# Autodesk Inventor assembly: PBM
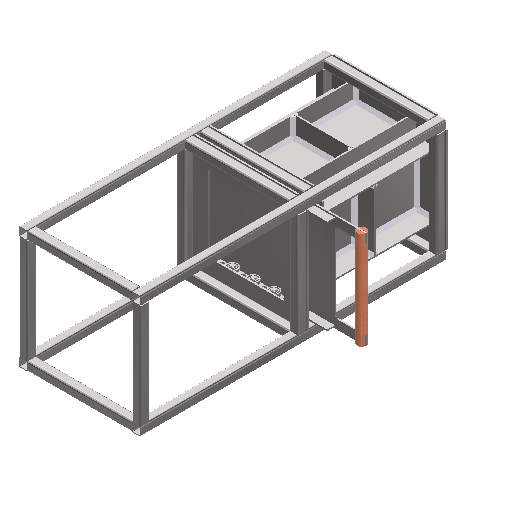
[picture p0: Inventor's stored thumbnail of the model, 512x512]
Saved by Autodesk Inventor 2025.3 (Build 293356000, 356)
## iProperties
Created: 2024-06-07
Part Number: PBM
Document SubType Name: Weldment
Designer: teiko
Weld Material: Welded Aluminum-6061
Author: teiko
## Documents named in this file (5)
- C:\Users\VICTUS\Documents\Inventor\ProjectBindMe\PBM.iam
- C:\Users\VICTUS\Documents\Inventor\ProjectBindMe\PBM-STR.iam
- C:\Users\VICTUS\Documents\Inventor\ProjectBindMe\PBM-CMP.iam
- C:\Users\VICTUS\Documents\Inventor\ProjectBindMe\PBM-EJT.iam
- C:\Users\VICTUS\Documents\Inventor\ProjectBindMe\complete structure.iam
## Components (4 placed, 4 different names)
1. PBM-STR:1 [sub-assembly] — Flush:1, Flush:2, Flush:3, Mate:1, Flush:4, Flush:5, Mate:2, Flush:6, Flush:7, Symmetry:1, Mate:3
2. PBM-CMP:1 [sub-assembly] — Mate:1, Flush:4, Flush:5, Symmetry:1
3. PBM-EJT:1 [sub-assembly] — Mate:2, Flush:6, Flush:7
4. complete structure:1 [sub-assembly] — Mate:3
## Relationships (11: Flush 7, Mate 3, Symmetry 1)
- Flush:1: PBM-STR:1
- Flush:2: PBM-STR:1
- Flush:3: PBM-STR:1
- Mate:1: PBM-STR:1 ↔ PBM-CMP:1
- Flush:4: PBM-STR:1 ↔ PBM-CMP:1
- Flush:5: PBM-STR:1 ↔ PBM-CMP:1
- Mate:2: PBM-STR:1 ↔ PBM-EJT:1
- Flush:6: PBM-STR:1 ↔ PBM-EJT:1
- Flush:7: PBM-STR:1 ↔ PBM-EJT:1
- Symmetry:1: PBM-STR:1 ↔ PBM-CMP:1
- Mate:3: PBM-STR:1 ↔ complete structure:1
